# Autodesk Inventor assembly: Assembly1
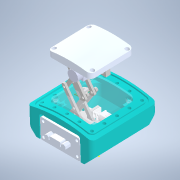
[picture p0: Inventor's stored thumbnail of the model, 180x180]
Saved by Autodesk Inventor 2020.1 (Build 241239000, 239)
## iProperties
Created: 2019-10-17
Part Number: Assembly1
Document SubType Name: Assembly
Designer: jesse
Author: jesse
## Documents named in this file (9)
- C:\Users\jesse\Desktop\rocksat_2020_model\Port Cover Assembly.iam
- C:\Users\jesse\Desktop\rocksat_2020_model\MultipurposePort-Released_withSTL\Assembly Multipurpose Port.iam
- C:\Users\jesse\Desktop\rocksat_2020_model\n20-micro-metal-gearmotor-1.snapshot.2\n20 motor.iam
- C:\Users\jesse\Desktop\rocksat_2020_model\camera.ipt
- C:\Users\jesse\Desktop\rocksat_2020_model\s_arm.ipt
- C:\Users\jesse\Desktop\rocksat_2020_model\s_support.ipt
- C:\Users\jesse\Desktop\rocksat_2020_model\MultipurposePort-Released_withSTL\ME112673.ipt
- C:\Users\jesse\Desktop\robotux cad 2020\adapter.ipt
- C:\Users\jesse\Desktop\rocksat_2020_model\s_support_bottom.ipt
## Components (16 placed, 8 different names)
1. Assembly Multipurpose Port:1 [sub-assembly] — Mate:11, Mate:12, Mate:15, Flush:9, Flush:10, Mate:22, Mate:23, Mate:32
2. n20 motor:1 [sub-assembly] — Mate:22, Flush:11, Mate:33
3. camera:1 — Mate:13, Flush:5, Flush:6, Flush:7
4. s_arm:1 — Rotational:1, Mate:6, Mate:21, Mate:26
5. s_arm:2 — Rotational:1, Mate:7, Mate:8, Mate:25, Mate:29
6. s_support:3 — Mate:9, Mate:10, Mate:31, Mate:32
7. s_arm:3 — Mate:6, Mate:31
8. s_arm:4 — Mate:7, Mate:8, Mate:9
9. ME112673:1 — Mate:10, Mate:11, Mate:12, Mate:13, Flush:5, Flush:6, Mate:14, Flush:8, Mate:15
10. camera:2 — Mate:14, Flush:7, Flush:8
11. adapter:1 — Flush:9, Flush:10
12. s_arm:5 — Mate:21, Mate:28
13. s_arm:6 — Mate:27
14. s_arm:7
15. s_arm:8
16. s_support_bottom:1 — Mate:23, Mate:25, Mate:26, Mate:27, Mate:28, Mate:29, Flush:11, Mate:33
## Relationships (35: Mate 24, Flush 7, RevoluteJoint 4)
- Rotational:1 [RevoluteJoint]: s_arm:1 ↔ s_arm:2
- [RevoluteJoint]: s_arm:3 ↔ s_arm:4
- Mate:6: s_arm:1 ↔ s_arm:3
- Mate:7: s_arm:2 ↔ s_arm:4
- Mate:8: s_arm:2 ↔ s_arm:4
- Mate:9: s_support:3 ↔ s_arm:4
- Mate:10: s_support:3 ↔ ME112673:1
- Mate:11: Assembly Multipurpose Port:1 ↔ ME112673:1
- Mate:12: Assembly Multipurpose Port:1 ↔ ME112673:1
- Mate:13: camera:1 ↔ ME112673:1
- Flush:5: camera:1 ↔ ME112673:1
- Flush:6 (-29.0068 mm): camera:1 ↔ ME112673:1
- Mate:14: ME112673:1 ↔ camera:2
- Flush:7: camera:1 ↔ camera:2
- Flush:8: ME112673:1 ↔ camera:2
- Mate:15: Assembly Multipurpose Port:1 ↔ ME112673:1
- Flush:9: Assembly Multipurpose Port:1 ↔ adapter:1
- Flush:10: Assembly Multipurpose Port:1 ↔ adapter:1
- [RevoluteJoint]: s_arm:5 ↔ s_arm:6
- [RevoluteJoint]: s_arm:7 ↔ s_arm:8
- [Mate]: s_arm:5 ↔ s_arm:7
- [Mate]: s_arm:6 ↔ s_arm:8
- [Mate]: s_arm:6 ↔ s_arm:8
- Mate:21: s_arm:1 ↔ s_arm:5
- Mate:22: Assembly Multipurpose Port:1 ↔ n20 motor:1
- Mate:23: Assembly Multipurpose Port:1 ↔ s_support_bottom:1
- Mate:25: s_arm:2 ↔ s_support_bottom:1
- Mate:26: s_arm:1 ↔ s_support_bottom:1
- Mate:27: s_arm:6 ↔ s_support_bottom:1
- Mate:28: s_arm:5 ↔ s_support_bottom:1
- Mate:29: s_arm:2 ↔ s_support_bottom:1
- Flush:11: n20 motor:1 ↔ s_support_bottom:1
- Mate:31: s_support:3 ↔ s_arm:3
- Mate:32: Assembly Multipurpose Port:1 ↔ s_support:3
- Mate:33: n20 motor:1 ↔ s_support_bottom:1
## Named parameters: support_length = 58.42 mm, s_arm_length = 58.42 mm, d17_d2 = 0 mm, d18_d3 = 67.671716 deg, d41_d2 = 0 mm, d42_d3 = -112.328284 deg, d43_d17_d2 = 0 mm, d44_d18_d3 = 67.671716 deg, d45_d21 = 0 mm, d46_d22 = 0 mm, d47_d23 = 0 mm
